# Autodesk Inventor assembly: bed
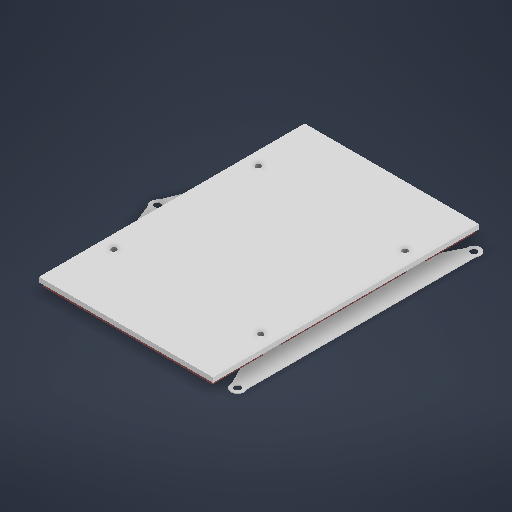
[picture p0: Inventor's stored thumbnail of the model, 512x512]
Saved by Autodesk Inventor 2025 (Build 290162000, 162)
## iProperties
Created: 2024-06-24
Part Number: bed
Document SubType Name: Assembly
Designer: Windows 7 was better
Author: Windows 7 was better
## Documents named in this file (4)
- C:\Users\Windows 7 was better\Documents\GitHub\ReplicatorPlusConversion\CAD\Inventor\bed-small.iam
- C:\Users\Windows 7 was better\Documents\GitHub\ReplicatorPlusConversion\CAD\Inventor\heater-small.ipt
- C:\Users\Windows 7 was better\Documents\GitHub\ReplicatorPlusConversion\CAD\Inventor\bed-small.ipt
- C:\Users\Windows 7 was better\Documents\GitHub\ReplicatorPlusConversion\CAD\Inventor\bed-plate-small.ipt
## Components (3 placed, 3 different names)
1. heater-small:1 — Flush:1
2. bed-small:1
3. bed-plate-small:1 — Flush:1
## Relationships (1: Flush 1)
- Flush:1: heater-small:1 ↔ bed-plate-small:1
